# Autodesk Inventor assembly: 1.2 ось
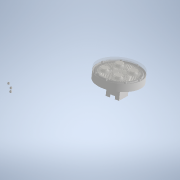
[picture p0: Inventor's stored thumbnail of the model, 180x180]
Saved by Autodesk Inventor 2021.2 (Build 252289000, 289)
## iProperties
Created: 2021-07-29
Part Number: 1.2 ось
Document SubType Name: Assembly
Designer: User
Author: User
## Documents named in this file (6)
- E:\Школа\Проекты\Аватар\3D-моделирование\1.2 ось\1.2 ось.iam
- E:\Школа\Проекты\Аватар\3D-моделирование\1.2 ось\Шар подшипника.ipt
- E:\Школа\Проекты\Аватар\3D-моделирование\1.2 ось\Солнце.ipt
- E:\Школа\Проекты\Аватар\3D-моделирование\1.2 ось\Основание с колесом нижнего редуктора\Основание с колесом нижнего редуктора.ipt
- E:\Школа\Проекты\Аватар\3D-моделирование\1.2 ось\Спутник.ipt
- E:\Школа\Проекты\Аватар\3D-моделирование\1.2 ось\Крышка.ipt
## Components (35 placed, 4 different names)
1. Шар подшипника:1 — Касательность:7
2. Цилиндрическое зубчатое зацепление1:2 — Заподлицо:4, Совмещение:1
3. Основание с колесом нижнего редуктора:1 — Заподлицо:4, Совмещение:1, Касательность:1, Касательность:2, Касательность:3, Касательность:4, Касательность:5, Касательность:6, Касательность:7, Касательность:8, Касательность:9, Касательность:10, Касательность:11, Касательность:12, Касательность:13, Касательность:14, Касательность:15, Касательность:16, Касательность:17, Касательность:18, Касательность:19, Касательность:20, Касательность:21, Касательность:22, Касательность:23, Касательность:24, Касательность:25, Заподлицо:5, Заподлицо:6, Заподлицо:7, Совмещение:2, Совмещение:3, Совмещение:4, Заподлицо:8, Совмещение:5, Совмещение:6, Совмещение:11
4. Шар подшипника:2 — Касательность:9
5. Шар подшипника:3 — Касательность:10
6. Шар подшипника:4 — Касательность:3
7. Шар подшипника:5 — Касательность:5
8. Шар подшипника:6 — Касательность:15
9. Шар подшипника:7 — Касательность:11
10. Шар подшипника:8 — Касательность:17
11. Шар подшипника:9 — Касательность:21
12. Шар подшипника:10 — Касательность:23
13. Шар подшипника:11 — Касательность:25
14. Шар подшипника:12
15. Шар подшипника:13 — Касательность:6
16. Шар подшипника:14 — Касательность:12
17. Шар подшипника:15 — Касательность:14
18. Шар подшипника:16
19. Шар подшипника:17
20. Шар подшипника:18 — Касательность:24
21. Шар подшипника:19 — Касательность:20
22. Шар подшипника:20 — Касательность:22
23. Шар подшипника:21 — Касательность:19
24. Шар подшипника:22 — Касательность:18
25. Шар подшипника:23 — Касательность:16
26. Шар подшипника:24 — Касательность:8
27. Шар подшипника:25 — Касательность:4
28. Шар подшипника:26 — Касательность:2
29. Шар подшипника:27 — Касательность:1
30. Шар подшипника:28 — Касательность:13
31. Цилиндрическое зубчатое зацепление1:3 — Заподлицо:6, Совмещение:2, Совмещение:7
32. Цилиндрическое зубчатое зацепление1:4 — Заподлицо:5, Совмещение:3, Совмещение:8
33. Цилиндрическое зубчатое зацепление1:5 — Заподлицо:7, Совмещение:4, Совмещение:9
34. Цилиндрическое зубчатое зацепление1:6 — Заподлицо:8, Совмещение:5, Совмещение:10
35. Крышка:1 — Совмещение:6, Совмещение:7, Совмещение:8, Совмещение:9, Совмещение:10, Совмещение:11
## Relationships (41: Tangent 25, Mate 11, Flush 5)
- Заподлицо:4 [Flush]: Цилиндрическое зубчатое зацепление1:2 ↔ Основание с колесом нижнего редуктора:1
- Совмещение:1 [Mate]: Цилиндрическое зубчатое зацепление1:2 ↔ Основание с колесом нижнего редуктора:1
- Касательность:1 [Tangent]: Основание с колесом нижнего редуктора:1 ↔ Шар подшипника:27
- Касательность:2 [Tangent]: Основание с колесом нижнего редуктора:1 ↔ Шар подшипника:26
- Касательность:3 [Tangent]: Основание с колесом нижнего редуктора:1 ↔ Шар подшипника:4
- Касательность:4 [Tangent]: Основание с колесом нижнего редуктора:1 ↔ Шар подшипника:25
- Касательность:5 [Tangent]: Основание с колесом нижнего редуктора:1 ↔ Шар подшипника:5
- Касательность:6 [Tangent]: Основание с колесом нижнего редуктора:1 ↔ Шар подшипника:13
- Касательность:7 [Tangent]: Шар подшипника:1 ↔ Основание с колесом нижнего редуктора:1
- Касательность:8 [Tangent]: Основание с колесом нижнего редуктора:1 ↔ Шар подшипника:24
- Касательность:9 [Tangent]: Основание с колесом нижнего редуктора:1 ↔ Шар подшипника:2
- Касательность:10 [Tangent]: Основание с колесом нижнего редуктора:1 ↔ Шар подшипника:3
- Касательность:11 [Tangent]: Основание с колесом нижнего редуктора:1 ↔ Шар подшипника:7
- Касательность:12 [Tangent]: Основание с колесом нижнего редуктора:1 ↔ Шар подшипника:14
- Касательность:13 [Tangent]: Основание с колесом нижнего редуктора:1 ↔ Шар подшипника:28
- Касательность:14 [Tangent]: Основание с колесом нижнего редуктора:1 ↔ Шар подшипника:15
- Касательность:15 [Tangent]: Основание с колесом нижнего редуктора:1 ↔ Шар подшипника:6
- Касательность:16 [Tangent]: Основание с колесом нижнего редуктора:1 ↔ Шар подшипника:23
- Касательность:17 [Tangent]: Основание с колесом нижнего редуктора:1 ↔ Шар подшипника:8
- Касательность:18 [Tangent]: Основание с колесом нижнего редуктора:1 ↔ Шар подшипника:22
- Касательность:19 [Tangent]: Основание с колесом нижнего редуктора:1 ↔ Шар подшипника:21
- Касательность:20 [Tangent]: Основание с колесом нижнего редуктора:1 ↔ Шар подшипника:19
- Касательность:21 [Tangent]: Основание с колесом нижнего редуктора:1 ↔ Шар подшипника:9
- Касательность:22 [Tangent]: Основание с колесом нижнего редуктора:1 ↔ Шар подшипника:20
- Касательность:23 [Tangent]: Основание с колесом нижнего редуктора:1 ↔ Шар подшипника:10
- Касательность:24 [Tangent]: Основание с колесом нижнего редуктора:1 ↔ Шар подшипника:18
- Касательность:25 [Tangent]: Основание с колесом нижнего редуктора:1 ↔ Шар подшипника:11
- Заподлицо:5 [Flush]: Основание с колесом нижнего редуктора:1 ↔ Цилиндрическое зубчатое зацепление1:4
- Заподлицо:6 [Flush]: Основание с колесом нижнего редуктора:1 ↔ Цилиндрическое зубчатое зацепление1:3
- Заподлицо:7 [Flush]: Основание с колесом нижнего редуктора:1 ↔ Цилиндрическое зубчатое зацепление1:5
- Совмещение:2 [Mate] (39.907 mm): Основание с колесом нижнего редуктора:1 ↔ Цилиндрическое зубчатое зацепление1:3
- Совмещение:3 [Mate] (39.907 mm): Основание с колесом нижнего редуктора:1 ↔ Цилиндрическое зубчатое зацепление1:4
- Совмещение:4 [Mate] (39.907 mm): Основание с колесом нижнего редуктора:1 ↔ Цилиндрическое зубчатое зацепление1:5
- Заподлицо:8 [Flush]: Основание с колесом нижнего редуктора:1 ↔ Цилиндрическое зубчатое зацепление1:6
- Совмещение:5 [Mate] (39.907 mm): Основание с колесом нижнего редуктора:1 ↔ Цилиндрическое зубчатое зацепление1:6
- Совмещение:6 [Mate]: Основание с колесом нижнего редуктора:1 ↔ Крышка:1
- Совмещение:7 [Mate]: Цилиндрическое зубчатое зацепление1:3 ↔ Крышка:1
- Совмещение:8 [Mate]: Цилиндрическое зубчатое зацепление1:4 ↔ Крышка:1
- Совмещение:9 [Mate]: Цилиндрическое зубчатое зацепление1:5 ↔ Крышка:1
- Совмещение:10 [Mate]: Цилиндрическое зубчатое зацепление1:6 ↔ Крышка:1
- Совмещение:11 [Mate] (2 mm): Основание с колесом нижнего редуктора:1 ↔ Крышка:1
